# Autodesk Inventor assembly: Bedienhebel
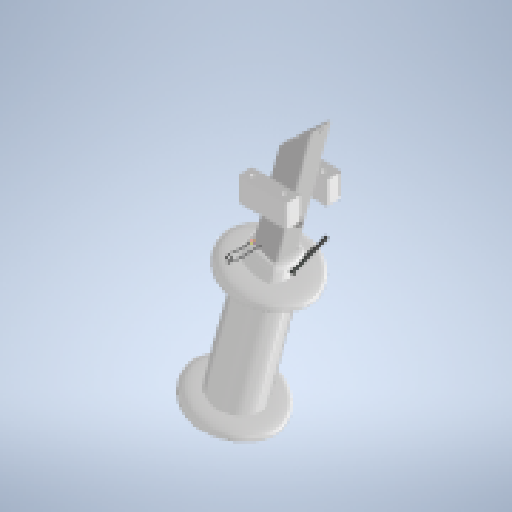
[picture p0: Inventor's stored thumbnail of the model, 512x512]
Saved by Autodesk Inventor 2025 (Build 290162010, 162A)
## iProperties
Created: 2024-11-27
Part Number: Bedienhebel
Document SubType Name: Assembly
Designer: Admin
Mass: 294.617 g
Surface Area: 838.082 cm^2
Volume: 215.984 cm^3
Density: 1.36406 g/cm^3
Author: Admin
## Documents named in this file (11)
- C:\Users\Admin\GIT\HDVKBM\CAD\Krandemonstrator\Bedienhebel.iam
- C:\Users\Admin\GIT\HDVKBM\CAD\Krandemonstrator\HebelhalterBlock.ipt
- C:\Users\Admin\GIT\HDVKBM\CAD\Krandemonstrator\HebelhalterBlockBlind.ipt
- C:\Users\Admin\GIT\HDVKBM\CAD\Krandemonstrator\ISO 12633-2 - 20x20x2 - 200.ipt
- C:\Users\Admin\GIT\HDVKBM\CAD\Krandemonstrator\Lagerhülse 6x4x0.ipt
- C:\Users\Admin\GIT\HDVKBM\CAD\Krandemonstrator\knaufErgo.ipt
- C:\Users\Admin\GIT\HDVKBM\CAD\Krandemonstrator\M3 Haken 40mm.ipt
- C:\Users\Admin\Documents\Inventor\Content Center Files\R2025\de-DE\ISO 4032(1)\ISO 4032 - M3DIN EN.ipt
- C:\Users\Admin\Documents\Inventor\Content Center Files\R2025\de-DE\ISO 10642(2)\ISO 10642  - M4  x  40.ipt
- C:\Users\Admin\Documents\Inventor\Content Center Files\R2025\de-DE\DIN EN ISO 7089\DIN EN ISO 7089 -  4.ipt
- C:\Users\Admin\Documents\Inventor\Content Center Files\R2025\de-DE\ISO 10642(2)\ISO 10642  - M3  x  30.ipt
## Components (11 placed, 10 different names)
1. HebelhalterBlock:1 — Starr:5
2. HebelhalterBlockBlind:1 — Starr:5, Drehbar:1
3. DIN EN ISO 10642 M4  x  40:1
4. ISO 12633-2 - 20x20x2 - 200:1 — Drehbar:1, Drehbar:2, Verschiebbar:1, Starr:7
5. DIN EN ISO 7089 4:1
6. DIN EN ISO 7089 4:2
7. Lagerhülse 6x4x0:1 — Drehbar:2
8. knaufErgo:1 — Verschiebbar:1
9. DIN EN ISO 10642 M3  x  30:1
10. M3 Haken 40mm:1 — Starr:7
11. DIN EN 24032 M3:1
## Relationships (9: WeldJoint 4, RevoluteJoint 2, Mate 1, TranslationJoint 1, Insert 1)
- [Mate]: HebelhalterBlock:1 ↔ DIN EN ISO 10642 M4  x  40:1
- [WeldJoint]: HebelhalterBlock:1 ↔ DIN EN ISO 7089 4:2
- Drehbar:1 [RevoluteJoint] (1 mm): HebelhalterBlockBlind:1 ↔ ISO 12633-2 - 20x20x2 - 200:1
- [WeldJoint]: HebelhalterBlockBlind:1 ↔ DIN EN ISO 7089 4:1
- Starr:5 [WeldJoint] (-22 mm): HebelhalterBlock:1 ↔ HebelhalterBlockBlind:1
- Drehbar:2 [RevoluteJoint]: ISO 12633-2 - 20x20x2 - 200:1 ↔ Lagerhülse 6x4x0:1
- Verschiebbar:1 [TranslationJoint]: ISO 12633-2 - 20x20x2 - 200:1 ↔ knaufErgo:1
- Starr:7 [WeldJoint]: ISO 12633-2 - 20x20x2 - 200:1 ↔ M3 Haken 40mm:1
- [Insert]: ISO 12633-2 - 20x20x2 - 200:1 ↔ DIN EN 24032 M3:1
